# Autodesk Inventor assembly: 38X18_frame
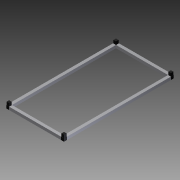
[picture p0: Inventor's stored thumbnail of the model, 180x180]
Saved by Autodesk Inventor 2011 SP1 (Build 150282100, 282)
## iProperties
Created: 2013-01-14
Part Number: 38X18_frame
Document SubType Name: Assembly
Designer: 351773
Author: 351773
## Documents named in this file (4)
- H:\GitHub\2013CAD\2013 robot\Common assemblies\prototype frame\38X18_frame.iam
- H:\GitHub\2013CAD\COTS parts\Plastic_Tubing_Connectors\3-way corner.ipt
- H:\GitHub\2013CAD\2013 robot\Common assemblies\prototype frame\1tube_16_frame.ipt
- H:\GitHub\2013CAD\2013 robot\Common assemblies\prototype frame\1tube_36_frame.ipt
## Components (8 placed, 3 different names)
1. 3-way corner:1 — Mate:1, Mate:2, Mate:3, Mate:4, Flush:1, Mate:5
2. 1tube_16_frame:1 — Flush:5, Mate:12, Mate:13, Mate:14
3. 1tube_36_frame:1 — Mate:8, Mate:9, Flush:3, Mate:15, Flush:6
4. 1tube_16_frame:2 — Mate:4, Flush:1, Mate:5, Mate:6, Flush:2, Mate:7
5. 1tube_36_frame:2 — Mate:1, Mate:2, Mate:3, Mate:10, Flush:4, Mate:11
6. 3-way corner:2 — Mate:6, Flush:2, Mate:7, Mate:8, Mate:9, Flush:3
7. 3-way corner:3 — Mate:14, Mate:15, Flush:6
8. 3-way corner:4 — Mate:10, Flush:4, Mate:11, Flush:5, Mate:12, Mate:13
## Relationships (21: Mate 15, Flush 6)
- Mate:1: 3-way corner:1 ↔ 1tube_36_frame:2
- Mate:2: 3-way corner:1 ↔ 1tube_36_frame:2
- Mate:3: 3-way corner:1 ↔ 1tube_36_frame:2
- Mate:4: 3-way corner:1 ↔ 1tube_16_frame:2
- Flush:1: 3-way corner:1 ↔ 1tube_16_frame:2
- Mate:5: 3-way corner:1 ↔ 1tube_16_frame:2
- Mate:6: 1tube_16_frame:2 ↔ 3-way corner:2
- Flush:2: 1tube_16_frame:2 ↔ 3-way corner:2
- Mate:7: 1tube_16_frame:2 ↔ 3-way corner:2
- Mate:8: 1tube_36_frame:1 ↔ 3-way corner:2
- Mate:9: 1tube_36_frame:1 ↔ 3-way corner:2
- Flush:3: 1tube_36_frame:1 ↔ 3-way corner:2
- Mate:10: 1tube_36_frame:2 ↔ 3-way corner:4
- Flush:4: 1tube_36_frame:2 ↔ 3-way corner:4
- Mate:11: 1tube_36_frame:2 ↔ 3-way corner:4
- Flush:5: 1tube_16_frame:1 ↔ 3-way corner:4
- Mate:12: 1tube_16_frame:1 ↔ 3-way corner:4
- Mate:13: 1tube_16_frame:1 ↔ 3-way corner:4
- Mate:14: 1tube_16_frame:1 ↔ 3-way corner:3
- Mate:15: 1tube_36_frame:1 ↔ 3-way corner:3
- Flush:6: 1tube_36_frame:1 ↔ 3-way corner:3
